# Autodesk Inventor assembly: Assembly_Cube_AlliedVision_Alvium_v3_2
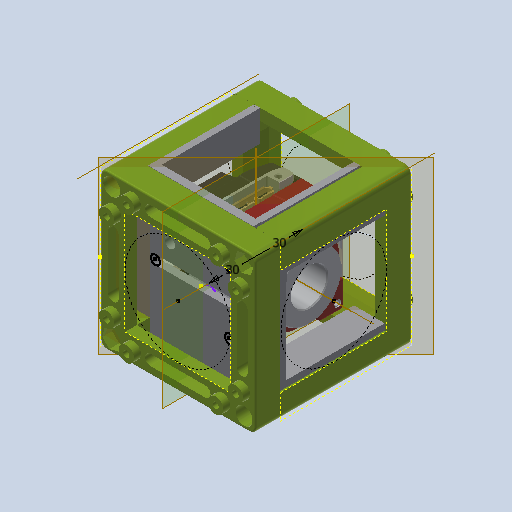
[picture p0: Inventor's stored thumbnail of the model, 512x512]
Saved by Autodesk Inventor 2022 (Build 260153000, 153)
## iProperties
Created: 2019-07-23
Part Number: Assembly_Cube_AlliedVision_Alvium_v3_2
Document SubType Name: Assembly
Designer: marsikovabarbora
Mass: 41.9543 g
Surface Area: 260.494 cm^2
Volume: 37.9382 cm^3
Density: 1.10586 g/cm^3
Author: marsikovabarbora
## Documents named in this file (4)
- C:\Users\UC2\Dropbox\UC2\02_CAD\INVENTOR\uc2_v3\Assembly_Cube_AlliedVision_Alvium_v3.iam
- C:\Users\UC2\Dropbox\UC2\02_CAD\INVENTOR\uc2_v3\00_Alvium_Step_USB90_S-Mount_ClosedHousing_2019-Mar-28.ipt
- C:\Users\UC2\Dropbox\UC2\02_CAD\INVENTOR\uc2_v3\20_Cube_insert_AlliedVision_Alvium_v3.ipt
- C:\Users\UC2\Dropbox\UC2\02_CAD\INVENTOR\uc2_v3\Assembly_Cube_empty_IM_v3.iam
## Components (3 placed, 3 different names)
1. Assembly_Cube_empty_IM_v3:1 [sub-assembly] — Mate:2, Mate:4, Mate:5
2. 00_Alvium_Step_USB90_S-Mount_ClosedHousing_2019-Mar-28:1 — Insert:1, Mate:1, Mate:2
3. 20_Cube_insert_AlliedVision_Alvium_v3:1 — Insert:1, Mate:1, Mate:4, Mate:5
## Relationships (5: Mate 4, Insert 1)
- Insert:1: 00_Alvium_Step_USB90_S-Mount_ClosedHousing_2019-Mar-28:1 ↔ 20_Cube_insert_AlliedVision_Alvium_v3:1
- Mate:1: 00_Alvium_Step_USB90_S-Mount_ClosedHousing_2019-Mar-28:1 ↔ 20_Cube_insert_AlliedVision_Alvium_v3:1
- Mate:2: Assembly_Cube_empty_IM_v3:1 ↔ 00_Alvium_Step_USB90_S-Mount_ClosedHousing_2019-Mar-28:1
- Mate:4: Assembly_Cube_empty_IM_v3:1 ↔ 20_Cube_insert_AlliedVision_Alvium_v3:1
- Mate:5: Assembly_Cube_empty_IM_v3:1 ↔ 20_Cube_insert_AlliedVision_Alvium_v3:1
